# Autodesk Inventor assembly: main_assembly
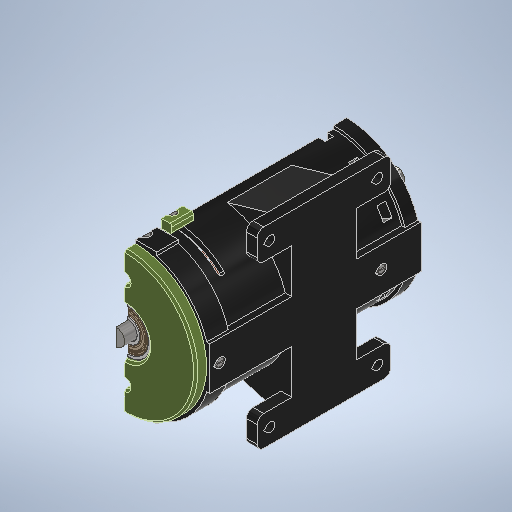
[picture p0: Inventor's stored thumbnail of the model, 512x512]
Saved by Autodesk Inventor 2025 (Build 290162000, 162)
## iProperties
Created: 2026-08-03
Part Number: main_assembly
Document SubType Name: Assembly
Designer: zzapa
Author: zzapa
## Documents named in this file (25)
- C:\Users\zzapa\Desktop\Projekty\elektronika\engine-project\model\assemblies\main_assembly.iam
- C:\Users\zzapa\Desktop\Projekty\elektronika\engine-project\model\parts\stator_metal.ipt
- C:\Users\zzapa\Desktop\Projekty\elektronika\engine-project\model\assemblies\magnet_ring_assembly.iam
- C:\Users\zzapa\Desktop\Projekty\elektronika\engine-project\model\parts\casing_cylindrical.ipt
- C:\Users\zzapa\Desktop\Projekty\elektronika\engine-project\model\parts\rotor_plastic.ipt
- C:\Users\zzapa\Desktop\Projekty\elektronika\engine-project\model\assemblies\rotor_core.iam
- C:\Users\zzapa\Desktop\Projekty\elektronika\engine-project\model\parts\shaft.ipt
- C:\Users\zzapa\Documents\Inventor\Content Center Files\R2025\pl-PL\GB 809-88 A\Nut GB 809 A M2,5 x 6.ipt
- C:\Users\zzapa\Documents\Inventor\Content Center Files\R2025\pl-PL\CNS 4355\CNS 4355 - M 2 x 6.ipt
- C:\Users\zzapa\Desktop\Projekty\elektronika\engine-project\model\parts\shaft_lock_1.ipt
- C:\Users\zzapa\Documents\Inventor\Content Center Files\R2025\pl-PL\GB 809-88 A\Nut GB 809 A M2 x 3.ipt
- C:\Users\zzapa\Documents\Inventor\Content Center Files\R2025\pl-PL\CNS 4355\CNS 4355 - M 2 x 8.ipt
- C:\Users\zzapa\Desktop\Projekty\elektronika\engine-project\model\parts\shaft_lock_2.ipt
- C:\Users\zzapa\Desktop\Projekty\elektronika\engine-project\model\assemblies\commutator_assembly.iam
- C:\Users\zzapa\Desktop\Projekty\elektronika\engine-project\model\parts\608zz.ipt
- C:\Users\zzapa\Desktop\Projekty\elektronika\engine-project\model\parts\sleeve.ipt
- C:\Users\zzapa\Desktop\Projekty\elektronika\engine-project\model\parts\rotor_sleeve.ipt
- C:\Users\zzapa\Desktop\Projekty\elektronika\engine-project\model\parts\carbon_brush_batt.ipt
- C:\Users\zzapa\Desktop\Projekty\elektronika\engine-project\model\parts\brush_cart_outer_holder.ipt
- C:\Users\zzapa\Desktop\Projekty\elektronika\engine-project\model\parts\brush_holder_batt.ipt
- C:\Users\zzapa\Desktop\Projekty\elektronika\engine-project\model\parts\single_coil.ipt
- C:\Users\zzapa\Desktop\Projekty\elektronika\engine-project\model\parts\name_plate.ipt
- C:\Users\zzapa\Desktop\Projekty\elektronika\engine-project\model\parts\back_sleeve.ipt
- C:\Users\zzapa\Documents\Inventor\Content Center Files\R2025\pl-PL\DIN 472(1)\DIN 472 - 22 x 1.ipt
- C:\Users\zzapa\Desktop\Projekty\elektronika\engine-project\model\parts\brush_spring.ipt
## Components (74 placed, 24 different names)
1. casing_cylindrical:1 — Zestawiające:3, Zestawiające:70, Zestawiające:81, Zestawiające:83, Zestawiające:84, Zestawiające:85, Zestawiające:86, Zestawiające:92, Zestawiające:93, Zestawiające:97, Zestawiające:98, Zestawiające:102, Zestawiające:104, Zestawiające:105, Zestawiające:108, Zestawiające:116, Kątowe:21, Zestawiające:117, Zestawiające:120, Wstawiające:6, Zestawiające:125, Zestawiające:126, Zestawiające:127, Zestawiające:129, Zestawiające:131
2. stator_metal:1 — Zestawiające:1, Zestawiające:81, Zestawiające:82
3. magnet_ring_assembly:1 [sub-assembly] — Zestawiające:78, Zestawiające:79, Zestawiające:82
4. shaft:1 — Zestawiające:6, Zestawiające:28, Styczny:1, Styczny:2, Zestawiające:50, Zestawiające:66, Zestawiające:71, Zestawiające:79, Zestawiające:87, Zestawiające:95, Zestawiające:111, Zestawiające:115, Równoległe:24, Kątowe:23
5. rotor_plastic:1 — Zestawiające:4, Zestawiające:7, Zestawiające:8, Zestawiające:9, Zestawiające:10, Równoległe:1, Równoległe:2, Równoległe:3, Równoległe:4, Zestawiające:31, Zestawiające:40, Zestawiające:41, Zestawiające:42, Zestawiające:43, Zestawiające:44, Równoległe:5, Równoległe:6, Równoległe:7, Równoległe:8, Kątowe:13, Symetria:1, Zestawiające:118, Zestawiające:119
6. shaft_lock_1:1 — Zestawiające:28, Zestawiające:30, Zestawiające:31, Zestawiające:32, Zestawiające:33, Zestawiające:34, Zestawiające:35, Zestawiające:36, Zestawiające:37, Zestawiające:38, Zestawiające:39, Zestawiające:40, Zestawiające:45, Zestawiające:46, Równoległe:9, Równoległe:10, Zestawiające:88
7. shaft_lock_2:1 — Zestawiające:50, Zestawiające:51, Zestawiające:53, Zestawiające:54, Równoległe:12, Równoległe:13, Zestawiające:58, Zestawiające:59, Zestawiające:60, Zestawiające:61, Zestawiające:62, Zestawiające:63, Zestawiające:64, Zestawiające:65, Zestawiające:67
8. rotor_core:1 [sub-assembly] — Zestawiające:5, Zestawiające:30, Zestawiające:67, Symetria:1, Kątowe:22
9. rotor_sleeve:1 — Zestawiające:87, Zestawiające:88, Kątowe:24
10. name_plate:1 — Zestawiające:103, Wstawiające:5, Zestawiające:106, Zestawiające:107, Zestawiające:108, Równoległe:24, Zestawiające:120
11. sleeve:1 — Zestawiające:97, Zestawiające:98, Zestawiające:99, Zestawiające:100, Zestawiające:101, Równoległe:21, Równoległe:22, Równoległe:23, Zestawiające:102, Zestawiające:103, Zestawiające:109, Zestawiające:113, Zestawiające:114, Zestawiające:119
12. 608zz:1 — Zestawiające:71, Kątowe:18, Zestawiające:109
13. DIN 472 22 x 1:1 — Zestawiające:113, Zestawiające:114, Kątowe:25
14. back_sleeve:1 — Zestawiające:115, Zestawiające:116, Kątowe:21, Zestawiające:117, Równoległe:25, Zestawiające:121, Zestawiające:122, Zestawiające:123, Zestawiające:124, Równoległe:26, Równoległe:27, Równoległe:28, Równoległe:29
15. 608zz:2 — Zestawiające:111, Równoległe:25, Kątowe:26
16. commutator_assembly:1 [sub-assembly] — Zestawiające:66, Styczny:3, Kątowe:20, Zestawiające:118
17. sprezyna_sprzeglo:1 — Zestawiające:132, Zestawiające:134, Kątowe:70, Kątowe:72
18. sprezyna_sprzeglo:2 — Zestawiające:133, Zestawiające:135, Kątowe:71
19. Nut GB/T 809-1988 Type A M2,5x6:1 — Kątowe:3, Zestawiające:7, Równoległe:3
20. Nut GB/T 809-1988 Type A M2,5x6:2 — Kątowe:4, Zestawiające:9, Równoległe:1
21. Nut GB/T 809-1988 Type A M2,5x6:3 — Kątowe:5, Zestawiające:8, Równoległe:2, Zestawiające:51
22. Nut GB/T 809-1988 Type A M2,5x6:4 — Kątowe:6, Zestawiające:10, Równoległe:4
23. Nut GB/T 809-1988 Type A M2,5x6:6 — Zestawiające:42, Równoległe:7, Kątowe:64
24. Nut GB/T 809-1988 Type A M2,5x6:7 — Zestawiające:44, Równoległe:6, Kątowe:63
25. Nut GB/T 809-1988 Type A M2,5x6:9 — Zestawiające:41, Równoległe:8, Kątowe:62
26. Nut GB/T 809-1988 Type A M2,5x6:8 — Zestawiające:43, Równoległe:5, Kątowe:61
27. Nut GB/T 809-1988 Type A M2x3:1 — Zestawiające:45, Równoległe:10, Zestawiające:47, Kątowe:60
28. Nut GB/T 809-1988 Type A M2x3:2 — Zestawiające:46, Równoległe:9, Zestawiające:48, Kątowe:59
29. Nut GB/T 809-1988 Type A M2x3:3 — Zestawiające:53, Równoległe:13, Zestawiające:57, Kątowe:58
30. Nut GB/T 809-1988 Type A M2x3:4 — Zestawiające:54, Równoległe:12, Zestawiające:56, Kątowe:57
31. Nut GB/T 809-1988 Type A M2x3:10 — Zestawiające:99, Równoległe:23, Kątowe:56
32. Nut GB/T 809-1988 Type A M2x3:11 — Zestawiające:100, Równoległe:22, Kątowe:55
33. Nut GB/T 809-1988 Type A M2x3:12 — Zestawiające:101, Równoległe:21, Kątowe:54
34. Nut GB/T 809-1988 Type A M2x3:13 — Zestawiające:123, Równoległe:28, Zestawiające:130, Kątowe:53
35. Nut GB/T 809-1988 Type A M2x3:14 — Zestawiające:124, Równoległe:26, Zestawiające:128, Kątowe:52
36. Nut GB/T 809-1988 Type A M2x3:15 — Zestawiające:122, Równoległe:27, Kątowe:51
37. Nut GB/T 809-1988 Type A M2x3:16 — Zestawiające:121, Równoległe:29, Kątowe:65
38. CNS 4355 M 2 x 6:5 — Zestawiające:32, Zestawiające:36, Kątowe:50
39. CNS 4355 M 2 x 6:6 — Zestawiające:35, Zestawiające:39, Kątowe:49
40. CNS 4355 M 2 x 6:7 — Zestawiające:34, Zestawiające:38, Kątowe:48
41. CNS 4355 M 2 x 6:8 — Zestawiające:33, Zestawiające:37, Kątowe:47
42. CNS 4355 M 2 x 8:1 — Zestawiające:48, Równoległe:11, Kątowe:46
43. CNS 4355 M 2 x 8:2 — Zestawiające:47, Zestawiające:49, Kątowe:45
44. CNS 4355 M 2 x 8:3 — Zestawiające:55, Zestawiające:57, Kątowe:44
45. CNS 4355 M 2 x 8:4 — Równoległe:14, Zestawiające:56, Kątowe:43
46. CNS 4355 M 2 x 6:9 — Zestawiające:60, Zestawiające:63, Kątowe:67
47. CNS 4355 M 2 x 6:10 — Zestawiające:61, Zestawiające:64, Kątowe:41
48. CNS 4355 M 2 x 6:11 — Zestawiające:59, Zestawiające:65, Kątowe:68
49. CNS 4355 M 2 x 6:12 — Zestawiające:58, Zestawiające:62, Kątowe:39
50. CNS 4355 M 2 x 8:5 — Zestawiające:83, Zestawiające:84, Kątowe:38
51. CNS 4355 M 2 x 8:6 — Zestawiające:85, Zestawiające:86, Kątowe:37
52. CNS 4355 M 2 x 8:9 — Wstawiające:5, Kątowe:36
53. CNS 4355 M 2 x 8:10 — Zestawiające:104, Zestawiające:106, Kątowe:35
54. CNS 4355 M 2 x 8:11 — Zestawiające:105, Zestawiające:107, Kątowe:66
55. CNS 4355 M 2 x 6:13 — Wstawiające:6, Kątowe:33
56. CNS 4355 M 2 x 6:14 — Zestawiające:127, Zestawiające:128, Kątowe:32
57. CNS 4355 M 2 x 6:15 — Zestawiające:129, Zestawiające:130, Kątowe:31
58. CNS 4355 M 2 x 6:16 — Zestawiające:125, Zestawiające:126, Kątowe:30
59. single_coil:1 — Zestawiające:95, Zestawiające:96, Równoległe:20
60. single_coil:2
61. single_coil:3
62. single_coil:4
63. single_coil:5
64. single_coil:6
65. brush_holder_batt:1 — Zestawiające:89, Równoległe:18, Zestawiające:91, Zestawiające:131, Zestawiające:133, Zestawiające:134, Zestawiające:135
66. brush_cart_outer_holder:1 — Zestawiające:90, Zestawiające:92, Zestawiające:93, Wstawiające:4
67. CNS 4355 M 2 x 8:7 — Wstawiające:4, Kątowe:29
68. Nut GB/T 809-1988 Type A M2x3:8 — Zestawiające:89, Równoległe:18, Zestawiające:90, Kątowe:28
69. carbon_brush_batt:1 — Zestawiające:91, Równoległe:19, Kątowe:27
70. brush_holder_batt:2 — Zestawiające:132
71. brush_cart_outer_holder:2
72. CNS 4355 M 2 x 8:8
73. Nut GB/T 809-1988 Type A M2x3:9
74. carbon_brush_batt:2
## Component patterns: (6 elements, first: single_coil:1), (2 elements, first: brush_holder_batt:1 + brush_cart_outer_holder:1 + CNS 4355 M 2 x 8:7 + Nut GB/T 809-1988 Type A M2x3:8 + carbon_brush_batt:1)
## Relationships (194: Mate 103, Angle 58, Flush 26, Tangent 3, Insert 3, Symmetry 1)
- Zestawiające:1 [Mate]: stator_metal:1
- Zestawiające:3 [Mate]: casing_cylindrical:1
- Zestawiające:4 [Mate]: rotor_plastic:1
- Zestawiające:5 [Mate]: rotor_core:1
- Zestawiające:6 [Mate]: shaft:1
- Kątowe:3 [Angle] (0 deg): Nut GB/T 809-1988 Type A M2,5x6:1
- Kątowe:4 [Angle] (0 deg): Nut GB/T 809-1988 Type A M2,5x6:2
- Kątowe:5 [Angle] (0 deg): Nut GB/T 809-1988 Type A M2,5x6:3
- Kątowe:6 [Angle] (0 deg): Nut GB/T 809-1988 Type A M2,5x6:4
- Zestawiające:7 [Mate]: rotor_plastic:1 ↔ Nut GB/T 809-1988 Type A M2,5x6:1
- Zestawiające:8 [Mate]: rotor_plastic:1 ↔ Nut GB/T 809-1988 Type A M2,5x6:3
- Zestawiające:9 [Mate]: rotor_plastic:1 ↔ Nut GB/T 809-1988 Type A M2,5x6:2
- Zestawiające:10 [Mate]: rotor_plastic:1 ↔ Nut GB/T 809-1988 Type A M2,5x6:4
- Równoległe:1 [Flush]: rotor_plastic:1 ↔ Nut GB/T 809-1988 Type A M2,5x6:2
- Równoległe:2 [Flush]: rotor_plastic:1 ↔ Nut GB/T 809-1988 Type A M2,5x6:3
- Równoległe:3 [Flush]: rotor_plastic:1 ↔ Nut GB/T 809-1988 Type A M2,5x6:1
- Równoległe:4 [Flush]: rotor_plastic:1 ↔ Nut GB/T 809-1988 Type A M2,5x6:4
- Zestawiające:28 [Mate]: shaft:1 ↔ shaft_lock_1:1
- Zestawiające:30 [Mate]: shaft_lock_1:1 ↔ rotor_core:1
- Zestawiające:31 [Mate]: rotor_plastic:1 ↔ shaft_lock_1:1
- Zestawiające:32 [Mate]: shaft_lock_1:1 ↔ CNS 4355 M 2 x 6:5
- Zestawiające:33 [Mate]: shaft_lock_1:1 ↔ CNS 4355 M 2 x 6:8
- Zestawiające:34 [Mate]: shaft_lock_1:1 ↔ CNS 4355 M 2 x 6:7
- Zestawiające:35 [Mate]: shaft_lock_1:1 ↔ CNS 4355 M 2 x 6:6
- Zestawiające:36 [Mate]: shaft_lock_1:1 ↔ CNS 4355 M 2 x 6:5
- Zestawiające:37 [Mate]: shaft_lock_1:1 ↔ CNS 4355 M 2 x 6:8
- Zestawiające:38 [Mate]: shaft_lock_1:1 ↔ CNS 4355 M 2 x 6:7
- Zestawiające:39 [Mate]: shaft_lock_1:1 ↔ CNS 4355 M 2 x 6:6
- Zestawiające:40 [Mate]: rotor_plastic:1 ↔ shaft_lock_1:1
- Zestawiające:41 [Mate]: rotor_plastic:1 ↔ Nut GB/T 809-1988 Type A M2,5x6:9
- Zestawiające:42 [Mate]: rotor_plastic:1 ↔ Nut GB/T 809-1988 Type A M2,5x6:6
- Zestawiające:43 [Mate]: rotor_plastic:1 ↔ Nut GB/T 809-1988 Type A M2,5x6:8
- Zestawiające:44 [Mate]: rotor_plastic:1 ↔ Nut GB/T 809-1988 Type A M2,5x6:7
- Równoległe:5 [Flush]: rotor_plastic:1 ↔ Nut GB/T 809-1988 Type A M2,5x6:8
- Równoległe:6 [Flush]: rotor_plastic:1 ↔ Nut GB/T 809-1988 Type A M2,5x6:7
- Równoległe:7 [Flush]: rotor_plastic:1 ↔ Nut GB/T 809-1988 Type A M2,5x6:6
- Równoległe:8 [Flush]: rotor_plastic:1 ↔ Nut GB/T 809-1988 Type A M2,5x6:9
- Kątowe:13 [Angle] (0 deg): rotor_plastic:1
- Zestawiające:45 [Mate]: shaft_lock_1:1 ↔ Nut GB/T 809-1988 Type A M2x3:1
- Zestawiające:46 [Mate]: shaft_lock_1:1 ↔ Nut GB/T 809-1988 Type A M2x3:2
- Równoległe:9 [Flush]: shaft_lock_1:1 ↔ Nut GB/T 809-1988 Type A M2x3:2
- Równoległe:10 [Flush]: shaft_lock_1:1 ↔ Nut GB/T 809-1988 Type A M2x3:1
- Zestawiające:47 [Mate]: Nut GB/T 809-1988 Type A M2x3:1 ↔ CNS 4355 M 2 x 8:2
- Zestawiające:48 [Mate]: Nut GB/T 809-1988 Type A M2x3:2 ↔ CNS 4355 M 2 x 8:1
- Kątowe:14 [Angle] (0 deg)
- Styczny:1 [Tangent]: shaft:1
- Kątowe:15 [Angle] (0 deg)
- Styczny:2 [Tangent]: shaft:1
- Zestawiające:49 [Mate]: CNS 4355 M 2 x 8:2
- Równoległe:11 [Flush]: CNS 4355 M 2 x 8:1
- Zestawiające:50 [Mate]: shaft:1 ↔ shaft_lock_2:1
- Zestawiające:51 [Mate]: shaft_lock_2:1 ↔ Nut GB/T 809-1988 Type A M2,5x6:3
- Zestawiające:53 [Mate]: shaft_lock_2:1 ↔ Nut GB/T 809-1988 Type A M2x3:3
- Zestawiające:54 [Mate]: shaft_lock_2:1 ↔ Nut GB/T 809-1988 Type A M2x3:4
- Równoległe:12 [Flush]: shaft_lock_2:1 ↔ Nut GB/T 809-1988 Type A M2x3:4
- Równoległe:13 [Flush]: shaft_lock_2:1 ↔ Nut GB/T 809-1988 Type A M2x3:3
- Równoległe:14 [Flush]: CNS 4355 M 2 x 8:4
- Zestawiające:55 [Mate]: CNS 4355 M 2 x 8:3
- Zestawiające:56 [Mate]: Nut GB/T 809-1988 Type A M2x3:4 ↔ CNS 4355 M 2 x 8:4
- Zestawiające:57 [Mate]: Nut GB/T 809-1988 Type A M2x3:3 ↔ CNS 4355 M 2 x 8:3
- Zestawiające:58 [Mate]: shaft_lock_2:1 ↔ CNS 4355 M 2 x 6:12
- Zestawiające:59 [Mate]: shaft_lock_2:1 ↔ CNS 4355 M 2 x 6:11
- Zestawiające:60 [Mate]: shaft_lock_2:1 ↔ CNS 4355 M 2 x 6:9
- Zestawiające:61 [Mate]: shaft_lock_2:1 ↔ CNS 4355 M 2 x 6:10
- Zestawiające:62 [Mate]: shaft_lock_2:1 ↔ CNS 4355 M 2 x 6:12
- Zestawiające:63 [Mate]: shaft_lock_2:1 ↔ CNS 4355 M 2 x 6:9
- Zestawiające:64 [Mate]: shaft_lock_2:1 ↔ CNS 4355 M 2 x 6:10
- Zestawiające:65 [Mate]: shaft_lock_2:1 ↔ CNS 4355 M 2 x 6:11
- Zestawiające:66 [Mate]: shaft:1 ↔ commutator_assembly:1
- Zestawiające:67 [Mate]: shaft_lock_2:1 ↔ rotor_core:1
- Zestawiające:70 [Mate]: casing_cylindrical:1
- Zestawiające:71 [Mate]: shaft:1 ↔ 608zz:1
- Kątowe:18 [Angle] (0 deg): 608zz:1
- Zestawiające:78 [Mate]: magnet_ring_assembly:1
- Zestawiające:79 [Mate]: magnet_ring_assembly:1 ↔ shaft:1
- Zestawiające:81 [Mate]: casing_cylindrical:1 ↔ stator_metal:1
- Zestawiające:82 [Mate]: stator_metal:1 ↔ magnet_ring_assembly:1
- Zestawiające:83 [Mate]: casing_cylindrical:1 ↔ CNS 4355 M 2 x 8:5
- Zestawiające:84 [Mate]: casing_cylindrical:1 ↔ CNS 4355 M 2 x 8:5
- Zestawiające:85 [Mate]: casing_cylindrical:1 ↔ CNS 4355 M 2 x 8:6
- Zestawiające:86 [Mate]: casing_cylindrical:1 ↔ CNS 4355 M 2 x 8:6
- Zestawiające:87 [Mate]: shaft:1 ↔ rotor_sleeve:1
- Zestawiające:88 [Mate]: shaft_lock_1:1 ↔ rotor_sleeve:1
- Zestawiające:89 [Mate]: brush_holder_batt:1 ↔ Nut GB/T 809-1988 Type A M2x3:8
- Równoległe:18 [Flush]: brush_holder_batt:1 ↔ Nut GB/T 809-1988 Type A M2x3:8
- Zestawiające:90 [Mate]: brush_cart_outer_holder:1 ↔ Nut GB/T 809-1988 Type A M2x3:8
- Zestawiające:91 [Mate]: brush_holder_batt:1 ↔ carbon_brush_batt:1
- Kątowe:19 [Angle] (0 deg)
- Styczny:3 [Tangent]: commutator_assembly:1
- Zestawiające:92 [Mate]: casing_cylindrical:1 ↔ brush_cart_outer_holder:1
- Zestawiające:93 [Mate]: casing_cylindrical:1 ↔ brush_cart_outer_holder:1
- Równoległe:19 [Flush]: carbon_brush_batt:1
- Wstawiające:4 [Insert]: brush_cart_outer_holder:1 ↔ CNS 4355 M 2 x 8:7
- Zestawiające:95 [Mate]: shaft:1 ↔ single_coil:1
- Zestawiające:96 [Mate]: single_coil:1
- Symetria:1 [Symmetry]: rotor_plastic:1 ↔ rotor_core:1
- Równoległe:20 [Flush]: single_coil:1
- Zestawiające:97 [Mate]: casing_cylindrical:1 ↔ sleeve:1
- Zestawiające:98 [Mate]: casing_cylindrical:1 ↔ sleeve:1
- Zestawiające:99 [Mate]: sleeve:1 ↔ Nut GB/T 809-1988 Type A M2x3:10
- Zestawiające:100 [Mate]: sleeve:1 ↔ Nut GB/T 809-1988 Type A M2x3:11
- Zestawiające:101 [Mate]: sleeve:1 ↔ Nut GB/T 809-1988 Type A M2x3:12
- Równoległe:21 [Flush]: sleeve:1 ↔ Nut GB/T 809-1988 Type A M2x3:12
- Równoległe:22 [Flush]: sleeve:1 ↔ Nut GB/T 809-1988 Type A M2x3:11
- Równoległe:23 [Flush]: sleeve:1 ↔ Nut GB/T 809-1988 Type A M2x3:10
- Zestawiające:102 [Mate]: casing_cylindrical:1 ↔ sleeve:1
- Zestawiające:103 [Mate]: name_plate:1 ↔ sleeve:1
- Wstawiające:5 [Insert]: name_plate:1 ↔ CNS 4355 M 2 x 8:9
- Zestawiające:104 [Mate]: casing_cylindrical:1 ↔ CNS 4355 M 2 x 8:10
- Zestawiające:105 [Mate]: casing_cylindrical:1 ↔ CNS 4355 M 2 x 8:11
- Zestawiające:106 [Mate]: name_plate:1 ↔ CNS 4355 M 2 x 8:10
- Zestawiające:107 [Mate]: name_plate:1 ↔ CNS 4355 M 2 x 8:11
- Zestawiające:108 [Mate]: casing_cylindrical:1 ↔ name_plate:1
- Zestawiające:109 [Mate]: sleeve:1 ↔ 608zz:1
- Kątowe:20 [Angle] (0 deg): commutator_assembly:1
- Zestawiające:111 [Mate]: shaft:1 ↔ 608zz:2
- Zestawiające:113 [Mate]: sleeve:1 ↔ DIN 472 22 x 1:1
- Zestawiające:114 [Mate]: sleeve:1 ↔ DIN 472 22 x 1:1
- Zestawiające:115 [Mate]: shaft:1 ↔ back_sleeve:1
- Zestawiające:116 [Mate]: casing_cylindrical:1 ↔ back_sleeve:1
- Równoległe:24 [Flush] (20 mm): shaft:1 ↔ name_plate:1
- Kątowe:21 [Angle] (0 deg): casing_cylindrical:1 ↔ back_sleeve:1
- Zestawiające:117 [Mate]: casing_cylindrical:1 ↔ back_sleeve:1
- Zestawiające:118 [Mate] (14 mm): rotor_plastic:1 ↔ commutator_assembly:1
- Zestawiające:119 [Mate] (16 mm): rotor_plastic:1 ↔ sleeve:1
- Kątowe:22 [Angle] (0 deg): rotor_core:1
- Kątowe:23 [Angle] (0 deg): shaft:1
- Kątowe:24 [Angle] (0 deg): rotor_sleeve:1
- Równoległe:25 [Flush] (1.5 mm): back_sleeve:1 ↔ 608zz:2
- Zestawiające:120 [Mate]: casing_cylindrical:1 ↔ name_plate:1
- Zestawiające:121 [Mate]: back_sleeve:1 ↔ Nut GB/T 809-1988 Type A M2x3:16
- Zestawiające:122 [Mate]: back_sleeve:1 ↔ Nut GB/T 809-1988 Type A M2x3:15
- Zestawiające:123 [Mate]: back_sleeve:1 ↔ Nut GB/T 809-1988 Type A M2x3:13
- Zestawiające:124 [Mate]: back_sleeve:1 ↔ Nut GB/T 809-1988 Type A M2x3:14
- Równoległe:26 [Flush]: back_sleeve:1 ↔ Nut GB/T 809-1988 Type A M2x3:14
- Równoległe:27 [Flush]: back_sleeve:1 ↔ Nut GB/T 809-1988 Type A M2x3:15
- Równoległe:28 [Flush]: back_sleeve:1 ↔ Nut GB/T 809-1988 Type A M2x3:13
- Równoległe:29 [Flush]: back_sleeve:1 ↔ Nut GB/T 809-1988 Type A M2x3:16
- Wstawiające:6 [Insert]: casing_cylindrical:1 ↔ CNS 4355 M 2 x 6:13
- Zestawiające:125 [Mate]: casing_cylindrical:1 ↔ CNS 4355 M 2 x 6:16
- Zestawiające:126 [Mate]: casing_cylindrical:1 ↔ CNS 4355 M 2 x 6:16
- Zestawiające:127 [Mate]: casing_cylindrical:1 ↔ CNS 4355 M 2 x 6:14
- Zestawiające:128 [Mate]: Nut GB/T 809-1988 Type A M2x3:14 ↔ CNS 4355 M 2 x 6:14
- Zestawiające:129 [Mate]: casing_cylindrical:1 ↔ CNS 4355 M 2 x 6:15
- Zestawiające:130 [Mate]: Nut GB/T 809-1988 Type A M2x3:13 ↔ CNS 4355 M 2 x 6:15
- Kątowe:25 [Angle] (0 deg): DIN 472 22 x 1:1
- Kątowe:26 [Angle] (0 deg): 608zz:2
- Zestawiające:131 [Mate]: casing_cylindrical:1 ↔ brush_holder_batt:1
- Kątowe:27 [Angle] (0 deg): carbon_brush_batt:1
- Kątowe:28 [Angle] (0 deg): Nut GB/T 809-1988 Type A M2x3:8
- Kątowe:29 [Angle] (0 deg): CNS 4355 M 2 x 8:7
- Kątowe:30 [Angle] (0 deg): CNS 4355 M 2 x 6:16
- Kątowe:31 [Angle] (0 deg): CNS 4355 M 2 x 6:15
- Kątowe:32 [Angle] (0 deg): CNS 4355 M 2 x 6:14
- Kątowe:33 [Angle] (0 deg): CNS 4355 M 2 x 6:13
- Kątowe:35 [Angle] (0 deg): CNS 4355 M 2 x 8:10
- Kątowe:36 [Angle] (0 deg): CNS 4355 M 2 x 8:9
- Kątowe:37 [Angle] (0 deg): CNS 4355 M 2 x 8:6
- Kątowe:38 [Angle] (0 deg): CNS 4355 M 2 x 8:5
- Kątowe:39 [Angle] (0 deg): CNS 4355 M 2 x 6:12
- Kątowe:41 [Angle] (0 deg): CNS 4355 M 2 x 6:10
- Kątowe:43 [Angle] (0 deg): CNS 4355 M 2 x 8:4
- Kątowe:44 [Angle] (0 deg): CNS 4355 M 2 x 8:3
- Kątowe:45 [Angle] (0 deg): CNS 4355 M 2 x 8:2
- Kątowe:46 [Angle] (0 deg): CNS 4355 M 2 x 8:1
- Kątowe:47 [Angle] (0 deg): CNS 4355 M 2 x 6:8
- Kątowe:48 [Angle] (0 deg): CNS 4355 M 2 x 6:7
- Kątowe:49 [Angle] (0 deg): CNS 4355 M 2 x 6:6
- Kątowe:50 [Angle] (0 deg): CNS 4355 M 2 x 6:5
- Kątowe:51 [Angle] (0 deg): Nut GB/T 809-1988 Type A M2x3:15
- Kątowe:52 [Angle] (0 deg): Nut GB/T 809-1988 Type A M2x3:14
- Kątowe:53 [Angle] (0 deg): Nut GB/T 809-1988 Type A M2x3:13
- Kątowe:54 [Angle] (0 deg): Nut GB/T 809-1988 Type A M2x3:12
- Kątowe:55 [Angle] (0 deg): Nut GB/T 809-1988 Type A M2x3:11
- Kątowe:56 [Angle] (0 deg): Nut GB/T 809-1988 Type A M2x3:10
- Kątowe:57 [Angle] (0 deg): Nut GB/T 809-1988 Type A M2x3:4
- Kątowe:58 [Angle] (0 deg): Nut GB/T 809-1988 Type A M2x3:3
- Kątowe:59 [Angle] (0 deg): Nut GB/T 809-1988 Type A M2x3:2
- Kątowe:60 [Angle] (0 deg): Nut GB/T 809-1988 Type A M2x3:1
- Kątowe:61 [Angle] (0 deg): Nut GB/T 809-1988 Type A M2,5x6:8
- Kątowe:62 [Angle] (0 deg): Nut GB/T 809-1988 Type A M2,5x6:9
- Kątowe:63 [Angle] (0 deg): Nut GB/T 809-1988 Type A M2,5x6:7
- Kątowe:64 [Angle] (0 deg): Nut GB/T 809-1988 Type A M2,5x6:6
- Kątowe:65 [Angle] (0 deg): Nut GB/T 809-1988 Type A M2x3:16
- Kątowe:66 [Angle] (0 deg): CNS 4355 M 2 x 8:11
- Kątowe:67 [Angle] (0 deg): CNS 4355 M 2 x 6:9
- Kątowe:68 [Angle] (0 deg): CNS 4355 M 2 x 6:11
- Zestawiające:132 [Mate]: sprezyna_sprzeglo:1 ↔ brush_holder_batt:2
- Zestawiające:133 [Mate]: sprezyna_sprzeglo:2 ↔ brush_holder_batt:1
- Zestawiające:134 [Mate]: sprezyna_sprzeglo:1 ↔ brush_holder_batt:1
- Zestawiające:135 [Mate]: sprezyna_sprzeglo:2 ↔ brush_holder_batt:1
- Kątowe:70 [Angle] (0 deg): sprezyna_sprzeglo:1
- Kątowe:71 [Angle] (0 deg): sprezyna_sprzeglo:2
- Kątowe:72 [Angle] (0 deg): sprezyna_sprzeglo:1
